# Autodesk Inventor assembly: Soporte_Laterales
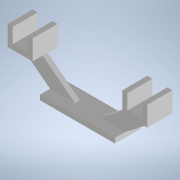
[picture p0: Inventor's stored thumbnail of the model, 180x180]
Saved by Autodesk Inventor 2020 (Build 240168000, 168)
## iProperties
Created: 2020-07-18
Part Number: Soporte_Laterales
Document SubType Name: Assembly
Designer: louis
Author: louis
## Documents named in this file (4)
- C:\Users\louis\Desktop\Robotica\Soporte_Laterales.iam
- C:\Users\louis\Desktop\Robotica\B_centro.ipt
- C:\Users\louis\Desktop\Robotica\Brazo_C.ipt
- C:\Users\louis\Desktop\Robotica\Tope_Centro.ipt
## Components (5 placed, 3 different names)
1. B_centro:1 — Coincidencia:1, Coincidencia:2, Nivelación:1, Coincidencia:7
2. Brazo_C:1 — Coincidencia:2, Nivelación:2, Coincidencia:4, Coincidencia:5, Coincidencia:7
3. Brazo_C:2 — Coincidencia:1, Nivelación:1, Nivelación:2, Nivelación:4, Coincidencia:6
4. Tope_Centro:1 — Coincidencia:3, Nivelación:3, Nivelación:4, Nivelación:5, Coincidencia:6
5. Tope_Centro:2 — Coincidencia:3, Coincidencia:4, Nivelación:3, Nivelación:5, Coincidencia:5
## Relationships (12: Mate 7, Flush 5)
- Coincidencia:1 [Mate]: B_centro:1 ↔ Brazo_C:2
- Coincidencia:2 [Mate]: B_centro:1 ↔ Brazo_C:1
- Nivelación:1 [Flush] (20 mm): B_centro:1 ↔ Brazo_C:2
- Nivelación:2 [Flush]: Brazo_C:1 ↔ Brazo_C:2
- Coincidencia:3 [Mate] (180 mm): Tope_Centro:1 ↔ Tope_Centro:2
- Coincidencia:4 [Mate]: Brazo_C:1 ↔ Tope_Centro:2
- Nivelación:3 [Flush]: Tope_Centro:1 ↔ Tope_Centro:2
- Nivelación:4 [Flush] (-20 mm): Brazo_C:2 ↔ Tope_Centro:1
- Nivelación:5 [Flush]: Tope_Centro:1 ↔ Tope_Centro:2
- Coincidencia:5 [Mate]: Brazo_C:1 ↔ Tope_Centro:2
- Coincidencia:6 [Mate]: Brazo_C:2 ↔ Tope_Centro:1
- Coincidencia:7 [Mate]: B_centro:1 ↔ Brazo_C:1
